# Autodesk Inventor assembly: Assembly4
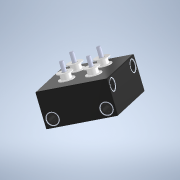
[picture p0: Inventor's stored thumbnail of the model, 180x180]
Saved by Autodesk Inventor 2021 (Build 250183000, 183)
## iProperties
Created: 2021-07-13
Part Number: Assembly4
Document SubType Name: Assembly
Designer: Michael Swaminathan
Author: Michael Swaminathan
## Documents named in this file (5)
- F:\Pattern Drawing Bot\Xy plotter mechanism\Assembly4.iam
- F:\Pattern Drawing Bot\Xy plotter mechanism\Central Portion.ipt
- F:\Pattern Drawing Bot\Xy plotter mechanism\Attachment Support.ipt
- F:\Pattern Drawing Bot\Xy plotter mechanism\Screw Support(Central Portion).ipt
- F:\Pattern Drawing Bot\Xy plotter mechanism\Rollers(2).ipt
## Components (17 placed, 4 different names)
1. Central Portion:1 — Rigid:1, Rigid:2, Rigid:3, Rigid:4, Rigid:5, Rigid:6, Rigid:7, Rigid:8, Rotational:1, Rotational:2, Rotational:3, Rotational:4, Rotational:5, Rotational:6, Rotational:7, Rotational:8
2. Attachment Support:1 — Rigid:1
3. Attachment Support:2 — Rigid:2
4. Attachment Support:3 — Rigid:4
5. Attachment Support:4 — Rigid:3
6. Attachment Support:5 — Rigid:6
7. Attachment Support:6 — Rigid:5
8. Attachment Support:7 — Rigid:8
9. Attachment Support:8 — Rigid:7
10. Screw Support(Central Portion):1 — Rotational:1
11. Screw Support(Central Portion):2 — Rotational:2
12. Screw Support(Central Portion):3 — Rotational:3
13. Screw Support(Central Portion):4 — Rotational:4
14. Rollers(2):1 — Rotational:5
15. Rollers(2):2 — Rotational:6
16. Rollers(2):3 — Rotational:7
17. Rollers(2):4 — Rotational:8
## Relationships (16: WeldJoint 8, RevoluteJoint 8)
- Rigid:1 [WeldJoint]: Central Portion:1 ↔ Attachment Support:1
- Rigid:2 [WeldJoint]: Central Portion:1 ↔ Attachment Support:2
- Rigid:3 [WeldJoint]: Central Portion:1 ↔ Attachment Support:4
- Rigid:4 [WeldJoint]: Central Portion:1 ↔ Attachment Support:3
- Rigid:5 [WeldJoint]: Central Portion:1 ↔ Attachment Support:6
- Rigid:6 [WeldJoint]: Central Portion:1 ↔ Attachment Support:5
- Rigid:7 [WeldJoint]: Central Portion:1 ↔ Attachment Support:8
- Rigid:8 [WeldJoint]: Central Portion:1 ↔ Attachment Support:7
- Rotational:1 [RevoluteJoint]: Central Portion:1 ↔ Screw Support(Central Portion):1
- Rotational:2 [RevoluteJoint]: Central Portion:1 ↔ Screw Support(Central Portion):2
- Rotational:3 [RevoluteJoint]: Central Portion:1 ↔ Screw Support(Central Portion):3
- Rotational:4 [RevoluteJoint]: Central Portion:1 ↔ Screw Support(Central Portion):4
- Rotational:5 [RevoluteJoint]: Central Portion:1 ↔ Rollers(2):1
- Rotational:6 [RevoluteJoint]: Central Portion:1 ↔ Rollers(2):2
- Rotational:7 [RevoluteJoint]: Central Portion:1 ↔ Rollers(2):3
- Rotational:8 [RevoluteJoint]: Central Portion:1 ↔ Rollers(2):4
